# Autodesk Inventor assembly: ChipMountAss
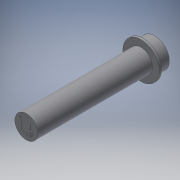
[picture p0: Inventor's stored thumbnail of the model, 180x180]
Saved by Autodesk Inventor 2019 (Build 230136000, 136)
## iProperties
Created: 2019-05-21
Part Number: ChipMountAss
Document SubType Name: Assembly
Designer: aorfi
Author: aorfi
## Documents named in this file (3)
- C:\Users\aorfi\Documents\IQC\ChipMountAssembly.iam
- C:\Users\aorfi\Documents\IQC\CustomParts\ChipMount.ipt
- C:\Users\aorfi\Documents\IQC\CustomParts\Chip.ipt
## Components (2 placed, 2 different names)
1. ChipMount:1 — Flush:1, Flush:2, Flush:3, Mate:1, Mate:2, Mate:3
2. Chip:1 — Mate:1, Mate:2, Mate:3
## Relationships (6: Flush 3, Mate 3)
- Flush:1: ChipMount:1
- Flush:2: ChipMount:1
- Flush:3: ChipMount:1
- Mate:1: ChipMount:1 ↔ Chip:1
- Mate:2: ChipMount:1 ↔ Chip:1
- Mate:3: ChipMount:1 ↔ Chip:1
